# Autodesk Inventor assembly: Сборка3
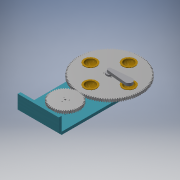
[picture p0: Inventor's stored thumbnail of the model, 180x180]
Saved by Autodesk Inventor 2018.3 (Build 223284000, 284)
## iProperties
Created: 2018-06-07
Part Number: Сборка3
Material: Типовые
Document SubType Name: Assembly
Designer: Leancher
Author: Leancher
## Documents named in this file (10)
- C:\Users\Leancher\My_projects\Al.Mechanic.CoffeeMachine\Сборка.iam
- C:\Users\Leancher\My_projects\Al.Mechanic.CoffeeMachine\Основание.ipt
- C:\Users\Leancher\My_projects\Al.Mechanic.CoffeeMachine\Ось.ipt
- C:\Users\Leancher\My_projects\Al.Mechanic.CoffeeMachine\Проставка шестерни.ipt
- C:\Users\Leancher\My_projects\Al.Mechanic.CoffeeMachine\Сборка\Мастер проектирования\Зубчатая передача1.iam
- C:\Users\Leancher\My_projects\Al.Mechanic.CoffeeMachine\Лейка.ipt
- C:\Users\Leancher\My_projects\Al.Mechanic.CoffeeMachine\Фильтр.ipt
- C:\Users\Leancher\My_projects\Al.Mechanic.CoffeeMachine\Фланец.ipt
- C:\Users\Leancher\My_projects\Al.Mechanic.CoffeeMachine\Держатель двигателя.ipt
- C:\Users\Leancher\My_projects\Al.Mechanic.CoffeeMachine\MotorNema14.ipt
## Components (12 placed, 9 different names)
1. Основание:1 — Совмещение:1
2. Ось:1 — Совмещение:1, Вставка:1, Вставка:2, Совмещение:3
3. Проставка шестерни:1 — Вставка:1, Совмещение:2, Совмещение:4
4. Зубчатая передача:1 [sub-assembly] — Совмещение:2, Совмещение:3, Совмещение:4, Вставка:3, Вставка:4, Вставка:5, Вставка:6, Вставка:7
5. Лейка:1 — Вставка:2
6. Фильтр:1 — Вставка:3
7. Фильтр:2 — Вставка:4
8. Фильтр:3 — Вставка:5
9. Фильтр:4 — Вставка:6
10. Фланец:1 — Вставка:7, Вставка:8
11. Держатель двигателя:1
12. MotorNema14:1 — Вставка:8
## Relationships (12: Insert 8, Mate 4)
- Совмещение:1 [Mate]: Основание:1 ↔ Ось:1
- Вставка:1 [Insert]: Ось:1 ↔ Проставка шестерни:1
- Вставка:2 [Insert]: Ось:1 ↔ Лейка:1
- Совмещение:2 [Mate]: Проставка шестерни:1 ↔ Зубчатая передача:1
- Совмещение:3 [Mate]: Ось:1 ↔ Зубчатая передача:1
- Совмещение:4 [Mate]: Проставка шестерни:1 ↔ Зубчатая передача:1
- Вставка:3 [Insert]: Зубчатая передача:1 ↔ Фильтр:1
- Вставка:4 [Insert]: Зубчатая передача:1 ↔ Фильтр:2
- Вставка:5 [Insert]: Зубчатая передача:1 ↔ Фильтр:3
- Вставка:6 [Insert]: Зубчатая передача:1 ↔ Фильтр:4
- Вставка:7 [Insert]: Зубчатая передача:1 ↔ Фланец:1
- Вставка:8 [Insert]: Фланец:1 ↔ MotorNema14:1
